# Autodesk Inventor assembly: arm-brack
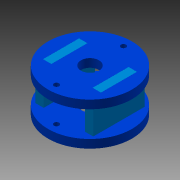
[picture p0: Inventor's stored thumbnail of the model, 180x180]
Saved by Autodesk Inventor 2013 (Build 170138000, 138)
## iProperties
Created: 2012-09-08
Part Number: arm-brack
Document SubType Name: Assembly
Designer: frankenteddy
Author: frankenteddy
## Documents named in this file (3)
- C:\Users\frankenteddy\Desktop\oshawatt1\arm-brack.iam
- C:\Users\frankenteddy\Desktop\oshawatt1\arm-bracket.ipt
- C:\Users\frankenteddy\Desktop\oshawatt1\arm-bracket-vert.ipt
## Components (4 placed, 2 different names)
1. arm-bracket:1 — Mate:1, Mate:2, Mate:3, Mate:8, Mate:9, Mate:10
2. arm-bracket-vert:1 — Mate:1, Mate:2, Mate:3
3. arm-bracket:2 — Mate:5, Mate:6, Mate:7
4. arm-bracket-vert:2 — Mate:5, Mate:6, Mate:7, Mate:8, Mate:9, Mate:10
## Relationships (9: Mate 9)
- Mate:1: arm-bracket:1 ↔ arm-bracket-vert:1
- Mate:2: arm-bracket:1 ↔ arm-bracket-vert:1
- Mate:3: arm-bracket:1 ↔ arm-bracket-vert:1
- Mate:5: arm-bracket:2 ↔ arm-bracket-vert:2
- Mate:6: arm-bracket:2 ↔ arm-bracket-vert:2
- Mate:7: arm-bracket:2 ↔ arm-bracket-vert:2
- Mate:8: arm-bracket:1 ↔ arm-bracket-vert:2
- Mate:9: arm-bracket:1 ↔ arm-bracket-vert:2
- Mate:10: arm-bracket:1 ↔ arm-bracket-vert:2
